# Autodesk Inventor assembly: Hexapod
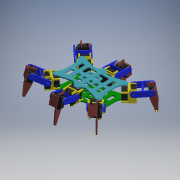
[picture p0: Inventor's stored thumbnail of the model, 180x180]
Saved by Autodesk Inventor 2017 (Build 210142000, 142)
## iProperties
Part Number: Hexapod
Document SubType Name: Assembly
Designer: Alexander Miller
Author: Alexander Miller
## Documents named in this file (6)
- D:\Daten\Documents\Git\Hexapod\3DParts\Hexapod.iam
- D:\Daten\Documents\Git\Hexapod\3DParts\Body_bottom.ipt
- D:\Daten\Documents\Git\Hexapod\3DParts\leg.iam
- D:\Daten\Documents\Git\Hexapod\3DParts\Body_top.ipt
- D:\Daten\Documents\Git\Hexapod\3DParts\Servo.ipt
- D:\Daten\Documents\Git\Hexapod\3DParts\Servo_arm.ipt
## Components (8 placed, 3 different names)
1. leg:1 [sub-assembly] — Rigid:3
2. leg:2 [sub-assembly] — Rigid:4
3. leg:3 [sub-assembly] — Rigid:2
4. leg:4 [sub-assembly] — Rigid:5
5. leg:5 [sub-assembly] — Rigid:1
6. leg:6 [sub-assembly] — Rigid:6
7. Body_top:1 — Rigid:1, Rigid:2, Rigid:3, Rigid:4, Rigid:5, Rigid:6, Mate:1, Flush:1, Flush:2
8. Body_bottom:1 — Mate:1, Flush:1, Flush:2
## Relationships (9: WeldJoint 6, Flush 2, Mate 1)
- Rigid:1 [WeldJoint]: leg:5 ↔ Body_top:1
- Rigid:2 [WeldJoint]: leg:3 ↔ Body_top:1
- Rigid:3 [WeldJoint]: leg:1 ↔ Body_top:1
- Rigid:4 [WeldJoint]: leg:2 ↔ Body_top:1
- Rigid:5 [WeldJoint]: leg:4 ↔ Body_top:1
- Rigid:6 [WeldJoint]: leg:6 ↔ Body_top:1
- Mate:1 (51 mm): Body_top:1 ↔ Body_bottom:1
- Flush:1: Body_top:1 ↔ Body_bottom:1
- Flush:2: Body_top:1 ↔ Body_bottom:1
## Named parameters: b_mat_thickness = 5 mm, s_height = 38 mm, s_shaft_height = 6 mm, sa_thickness = 2 mm
